# Autodesk Inventor assembly: RT_FRM_A_004_ElectricalFrame
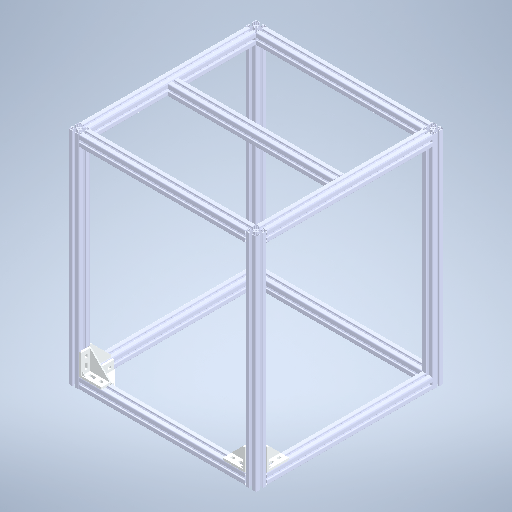
[picture p0: Inventor's stored thumbnail of the model, 512x512]
Saved by Autodesk Inventor 2025.3 (Build 293356000, 356)
## iProperties
Created: 2026-05-11
Part Number: RT_FRM_A_004_ElectricalFrame
Document SubType Name: Assembly
Designer: louis
Author: louis
## Documents named in this file (10)
- C:\Users\louis\OneDrive\Desktop\R_Trident\02_CAD\04_Subassemblies\RT_FRM_A_004_ElectricalFrame.iam
- C:\Users\louis\OneDrive\Desktop\R_Trident\02_CAD\01_Standard_Parts\Aluminium_Extrusions\4040x800_3619_20251007144627_4040.ipt
- C:\Users\louis\OneDrive\Desktop\R_Trident\02_CAD\01_Standard_Parts\Aluminium_Extrusions\4040x600_3619_20251007144627_4040.ipt
- C:\Users\louis\OneDrive\Desktop\R_Trident\02_CAD\01_Standard_Parts\3532_20210408113519_4080L + cover\3532_20210408113519_4080L + cover.iam
- C:\Users\louis\OneDrive\Desktop\R_Trident\02_CAD\04_Subassemblies\RT_FRM_A_004_ElectricalFrame\AIP\FEA\fg20fls1s.fins
- C:\Users\louis\OneDrive\Desktop\R_Trident\02_CAD\04_Subassemblies\RT_FRM_A_004_ElectricalFrame\AIP\FEA\fg20fls1s.fsat
- C:\Users\louis\OneDrive\Desktop\R_Trident\02_CAD\04_Subassemblies\RT_FRM_A_004_ElectricalFrame\AIP\FEA\fg20fls1s.ftes
- C:\Users\louis\OneDrive\Desktop\R_Trident\02_CAD\04_Subassemblies\RT_FRM_A_004_ElectricalFrame\AIP\FEA\fg20fls1s.fwiz
- C:\Users\louis\OneDrive\Desktop\R_Trident\02_CAD\04_Subassemblies\RT_FRM_A_004_ElectricalFrame\AIP\FEA\fg20fls68.fmsh
- C:\Users\louis\OneDrive\Desktop\R_Trident\02_CAD\04_Subassemblies\RT_FRM_A_004_ElectricalFrame\AIP\FEA\fg20fls69.fres
## Components (19 placed, 3 different names)
1. 4040x800_3619_20251007144627_4040:1 — Flush:2, Mate:2, Mate:4, Flush:6, Flush:12, Flush:13, Mate:11, Mate:13, Flush:19, Flush:24, Flush:25, Mate:24, Flush:37, Flush:39, Mate:28
2. 4040x800_3619_20251007144627_4040:2 — Flush:1, Flush:2, Flush:3, Mate:5, Mate:8, Flush:10, Flush:11, Mate:12, Flush:22, Flush:23
3. 4040x800_3619_20251007144627_4040:3 — Flush:3, Mate:3, Mate:6, Flush:5, Flush:14, Flush:15, Mate:10, Flush:18, Flush:20, Flush:26, Flush:27, Mate:17, Flush:34, Mate:20
4. 4040x800_3619_20251007144627_4040:4 — Flush:1, Mate:7, Mate:9, Flush:4, Flush:7, Flush:8, Flush:9, Flush:16, Flush:17, Flush:21, Flush:28
5. 4040x600_3619_20251007144627_4040:1 — Mate:2, Mate:3, Flush:5, Flush:13, Flush:14, Symmetry:1
6. 4040x600_3619_20251007144627_4040:2 — Mate:4, Mate:5, Flush:6, Flush:11, Flush:12, Mate:15, Flush:30, Symmetry:2, Symmetry:3
7. 4040x600_3619_20251007144627_4040:3 — Mate:6, Mate:7, Flush:4, Flush:9, Flush:15, Mate:14, Flush:29, Symmetry:3
8. 4040x600_3619_20251007144627_4040:4 — Mate:8, Mate:9, Flush:7, Flush:8, Flush:10, Symmetry:1
9. 4040x600_3619_20251007144627_4040:5 — Mate:10, Flush:16, Flush:20, Flush:27, Flush:28, Flush:35, Mate:19, Flush:36, Mate:22
10. 4040x600_3619_20251007144627_4040:6 — Mate:11, Flush:19, Flush:23, Flush:24, Symmetry:2, Flush:38, Mate:26, Mate:27
11. 4040x600_3619_20251007144627_4040:7 — Mate:13, Flush:18, Flush:25, Flush:26, Mate:18, Mate:21, Mate:23, Mate:25
12. 4040x600_3619_20251007144627_4040:8 — Mate:12, Flush:17, Flush:21, Flush:22
13. 4040x600_3619_20251007144627_4040:9 — Mate:14, Mate:15, Flush:29, Flush:30, Flush:31
14. 3532_20210408113519_4080L + cover:1 [sub-assembly] — Mate:17, Flush:34, Mate:18
15. 3532_20210408113519_4080L + cover:2 [sub-assembly] — Flush:35, Mate:19, Mate:20
16. 3532_20210408113519_4080L + cover:3 [sub-assembly] — Mate:21, Flush:36, Mate:22
17. 3532_20210408113519_4080L + cover:4 [sub-assembly] — Mate:23, Mate:24, Flush:37
18. 3532_20210408113519_4080L + cover:5 [sub-assembly] — Flush:39, Mate:27, Mate:28
19. 3532_20210408113519_4080L + cover:6 [sub-assembly] — Mate:25, Flush:38, Mate:26
## Relationships (69: Flush 39, Mate 27, Symmetry 3)
- Flush:1: 4040x800_3619_20251007144627_4040:2 ↔ 4040x800_3619_20251007144627_4040:4
- Flush:2: 4040x800_3619_20251007144627_4040:1 ↔ 4040x800_3619_20251007144627_4040:2
- Flush:3: 4040x800_3619_20251007144627_4040:2 ↔ 4040x800_3619_20251007144627_4040:3
- Mate:2: 4040x800_3619_20251007144627_4040:1 ↔ 4040x600_3619_20251007144627_4040:1
- Mate:3: 4040x800_3619_20251007144627_4040:3 ↔ 4040x600_3619_20251007144627_4040:1
- Mate:4: 4040x800_3619_20251007144627_4040:1 ↔ 4040x600_3619_20251007144627_4040:2
- Mate:5: 4040x800_3619_20251007144627_4040:2 ↔ 4040x600_3619_20251007144627_4040:2
- Mate:6: 4040x800_3619_20251007144627_4040:3 ↔ 4040x600_3619_20251007144627_4040:3
- Mate:7: 4040x800_3619_20251007144627_4040:4 ↔ 4040x600_3619_20251007144627_4040:3
- Mate:8: 4040x800_3619_20251007144627_4040:2 ↔ 4040x600_3619_20251007144627_4040:4
- Mate:9: 4040x800_3619_20251007144627_4040:4 ↔ 4040x600_3619_20251007144627_4040:4
- Flush:4: 4040x800_3619_20251007144627_4040:4 ↔ 4040x600_3619_20251007144627_4040:3
- Flush:5: 4040x800_3619_20251007144627_4040:3 ↔ 4040x600_3619_20251007144627_4040:1
- Flush:6: 4040x800_3619_20251007144627_4040:1 ↔ 4040x600_3619_20251007144627_4040:2
- Flush:7: 4040x800_3619_20251007144627_4040:4 ↔ 4040x600_3619_20251007144627_4040:4
- Flush:8: 4040x800_3619_20251007144627_4040:4 ↔ 4040x600_3619_20251007144627_4040:4
- Flush:9: 4040x800_3619_20251007144627_4040:4 ↔ 4040x600_3619_20251007144627_4040:3
- Flush:10: 4040x800_3619_20251007144627_4040:2 ↔ 4040x600_3619_20251007144627_4040:4
- Flush:11: 4040x800_3619_20251007144627_4040:2 ↔ 4040x600_3619_20251007144627_4040:2
- Flush:12: 4040x800_3619_20251007144627_4040:1 ↔ 4040x600_3619_20251007144627_4040:2
- Flush:13: 4040x800_3619_20251007144627_4040:1 ↔ 4040x600_3619_20251007144627_4040:1
- Flush:14: 4040x800_3619_20251007144627_4040:3 ↔ 4040x600_3619_20251007144627_4040:1
- Flush:15: 4040x800_3619_20251007144627_4040:3 ↔ 4040x600_3619_20251007144627_4040:3
- Mate:10: 4040x800_3619_20251007144627_4040:3 ↔ 4040x600_3619_20251007144627_4040:5
- Mate:11: 4040x800_3619_20251007144627_4040:1 ↔ 4040x600_3619_20251007144627_4040:6
- Mate:12: 4040x800_3619_20251007144627_4040:2 ↔ 4040x600_3619_20251007144627_4040:8
- Mate:13: 4040x800_3619_20251007144627_4040:1 ↔ 4040x600_3619_20251007144627_4040:7
- Flush:16: 4040x800_3619_20251007144627_4040:4 ↔ 4040x600_3619_20251007144627_4040:5
- Flush:17: 4040x800_3619_20251007144627_4040:4 ↔ 4040x600_3619_20251007144627_4040:8
- Flush:18: 4040x800_3619_20251007144627_4040:3 ↔ 4040x600_3619_20251007144627_4040:7
- Flush:19: 4040x800_3619_20251007144627_4040:1 ↔ 4040x600_3619_20251007144627_4040:6
- Flush:20: 4040x800_3619_20251007144627_4040:3 ↔ 4040x600_3619_20251007144627_4040:5
- Flush:21: 4040x800_3619_20251007144627_4040:4 ↔ 4040x600_3619_20251007144627_4040:8
- Flush:22: 4040x800_3619_20251007144627_4040:2 ↔ 4040x600_3619_20251007144627_4040:8
- Flush:23: 4040x800_3619_20251007144627_4040:2 ↔ 4040x600_3619_20251007144627_4040:6
- Flush:24: 4040x800_3619_20251007144627_4040:1 ↔ 4040x600_3619_20251007144627_4040:6
- Flush:25: 4040x800_3619_20251007144627_4040:1 ↔ 4040x600_3619_20251007144627_4040:7
- Flush:26: 4040x800_3619_20251007144627_4040:3 ↔ 4040x600_3619_20251007144627_4040:7
- Flush:27: 4040x800_3619_20251007144627_4040:3 ↔ 4040x600_3619_20251007144627_4040:5
- Flush:28: 4040x800_3619_20251007144627_4040:4 ↔ 4040x600_3619_20251007144627_4040:5
- Mate:14: 4040x600_3619_20251007144627_4040:3 ↔ 4040x600_3619_20251007144627_4040:9
- Mate:15: 4040x600_3619_20251007144627_4040:2 ↔ 4040x600_3619_20251007144627_4040:9
- Flush:29: 4040x600_3619_20251007144627_4040:3 ↔ 4040x600_3619_20251007144627_4040:9
- Flush:30: 4040x600_3619_20251007144627_4040:2 ↔ 4040x600_3619_20251007144627_4040:9
- Symmetry:1: 4040x600_3619_20251007144627_4040:1 ↔ 4040x600_3619_20251007144627_4040:4
- Symmetry:2: 4040x600_3619_20251007144627_4040:2 ↔ 4040x600_3619_20251007144627_4040:6
- Flush:31: 4040x600_3619_20251007144627_4040:9
- Flush:32
- Flush:33
- Symmetry:3: 4040x600_3619_20251007144627_4040:2 ↔ 4040x600_3619_20251007144627_4040:3
- Mate:16
- Mate:17: 4040x800_3619_20251007144627_4040:3 ↔ 3532_20210408113519_4080L + cover:1
- Flush:34: 4040x800_3619_20251007144627_4040:3 ↔ 3532_20210408113519_4080L + cover:1
- Mate:18: 4040x600_3619_20251007144627_4040:7 ↔ 3532_20210408113519_4080L + cover:1
- Flush:35: 4040x600_3619_20251007144627_4040:5 ↔ 3532_20210408113519_4080L + cover:2
- Mate:19: 4040x600_3619_20251007144627_4040:5 ↔ 3532_20210408113519_4080L + cover:2
- Mate:20: 4040x800_3619_20251007144627_4040:3 ↔ 3532_20210408113519_4080L + cover:2
- Mate:21: 4040x600_3619_20251007144627_4040:7 ↔ 3532_20210408113519_4080L + cover:3
- Flush:36: 4040x600_3619_20251007144627_4040:5 ↔ 3532_20210408113519_4080L + cover:3
- Mate:22: 4040x600_3619_20251007144627_4040:5 ↔ 3532_20210408113519_4080L + cover:3
- Mate:23: 4040x600_3619_20251007144627_4040:7 ↔ 3532_20210408113519_4080L + cover:4
- Mate:24: 4040x800_3619_20251007144627_4040:1 ↔ 3532_20210408113519_4080L + cover:4
- Flush:37: 4040x800_3619_20251007144627_4040:1 ↔ 3532_20210408113519_4080L + cover:4
- Mate:25: 4040x600_3619_20251007144627_4040:7 ↔ 3532_20210408113519_4080L + cover:6
- Flush:38: 4040x600_3619_20251007144627_4040:6 ↔ 3532_20210408113519_4080L + cover:6
- Mate:26: 4040x600_3619_20251007144627_4040:6 ↔ 3532_20210408113519_4080L + cover:6
- Flush:39: 4040x800_3619_20251007144627_4040:1 ↔ 3532_20210408113519_4080L + cover:5
- Mate:27: 4040x600_3619_20251007144627_4040:6 ↔ 3532_20210408113519_4080L + cover:5
- Mate:28: 4040x800_3619_20251007144627_4040:1 ↔ 3532_20210408113519_4080L + cover:5
## Named parameters: sa_0 = 10000, sa_1 = 20000
note: some values were not read from the file. Shown as the stored number, unit unknown: "sa_0", "sa_1".
